# Autodesk Inventor assembly: RC Car Assembly
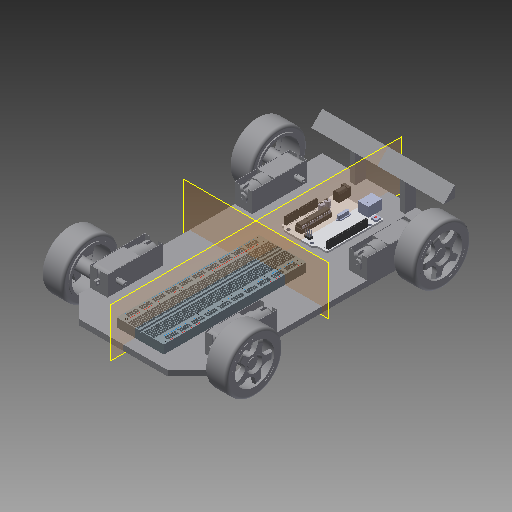
[picture p0: Inventor's stored thumbnail of the model, 512x512]
Saved by Autodesk Inventor 2019 (Build 230136000, 136)
## iProperties
Created: 2020-11-27
Part Number: RC Car Assembly
Document SubType Name: Assembly
Designer: wrong
Author: wrong
## Documents named in this file (12)
- C:\Users\wrong\Documents\Inventor\RC Car\RC Car Assembly.iam
- C:\Users\wrong\Documents\Inventor\RC Car\Arduino Uno.ipt
- C:\Users\wrong\Documents\Inventor\RC Car\BreadBoard.ipt
- C:\Users\wrong\Documents\Inventor\RC Car\Gear Motor.ipt
- C:\Users\wrong\Documents\Inventor\RC Car\RC Chassis.ipt
- C:\Users\wrong\Documents\Inventor\RC Car\Gear Motor_MIR.ipt
- C:\Users\wrong\Documents\Inventor\RC Car\Gear Motor_MIR1.ipt
- C:\Users\wrong\Documents\Inventor\RC Car\Gear Motor_MIR_MIR.ipt
- C:\Users\wrong\Documents\Inventor\RC Car\Wheel.ipt
- C:\Users\wrong\Documents\Inventor\RC Car\Wheel_MIR.ipt
- C:\Users\wrong\Documents\Inventor\RC Car\Wheel_MIR1.ipt
- C:\Users\wrong\Documents\Inventor\RC Car\Wheel_MIR_MIR.ipt
## Components (11 placed, 11 different names)
1. Arduino Uno:1 — Mate:4, Insert:1, Angle:1
2. BreadBoard:1 — Mate:2
3. RC Chassis:1 — Mate:2, Mate:4, Insert:1, Angle:1, Mate:5, Flush:1
4. Gear Motor:3 — Mate:5, Flush:1
5. Gear Motor_MIR:1
6. Gear Motor_MIR1:1
7. Gear Motor_MIR_MIR:1 — Mate:6, Mate:7, Tangent:1
8. Wheel:1 — Mate:6, Mate:7, Tangent:1
9. Wheel_MIR:1
10. Wheel_MIR1:1
11. Wheel_MIR_MIR:1
## Relationships (9: Mate 5, Insert 1, Angle 1, Flush 1, Tangent 1)
- Mate:2: BreadBoard:1 ↔ RC Chassis:1
- Mate:4: Arduino Uno:1 ↔ RC Chassis:1
- Insert:1: Arduino Uno:1 ↔ RC Chassis:1
- Angle:1 (0 deg): Arduino Uno:1 ↔ RC Chassis:1
- Mate:5: RC Chassis:1 ↔ Gear Motor:3
- Flush:1 (0.635 mm): RC Chassis:1 ↔ Gear Motor:3
- Mate:6: Gear Motor_MIR_MIR:1 ↔ Wheel:1
- Mate:7: Gear Motor_MIR_MIR:1 ↔ Wheel:1
- Tangent:1: Gear Motor_MIR_MIR:1 ↔ Wheel:1
